# Autodesk Inventor assembly: assembly
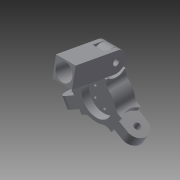
[picture p0: Inventor's stored thumbnail of the model, 180x180]
Saved by Autodesk Inventor 2014 SP2 (Build 180246200, 246)
## iProperties
Created: 2016-12-02
Part Number: assembly
Document SubType Name: Assembly
Designer: Justin B
Author: Justin B
## Documents named in this file (3)
- C:\Users\Justin B\Documents\Acoustic\assembly.iam
- C:\Users\Justin B\Documents\Acoustic\hub.ipt
- C:\Users\Justin B\Documents\Acoustic\spoke.ipt
## Components (2 placed, 2 different names)
1. hub:1 — Rotational:1
2. spoke:1 — Rotational:1
## Relationships (1: RevoluteJoint 1)
- Rotational:1 [RevoluteJoint] (-0.5 mm): hub:1 ↔ spoke:1
